# Autodesk Inventor assembly: mini Cryostat FOOT3
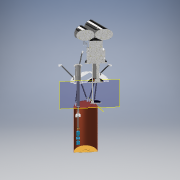
[picture p0: Inventor's stored thumbnail of the model, 180x180]
Saved by Autodesk Inventor 2018 (Build 220112000, 112)
## iProperties
Created: 2018-10-10
Part Number: mini Cryostat FOOT3
Document SubType Name: Assembly
Designer: Admin
Author: Admin
## Documents named in this file (11)
- C:\Users\Admin\Documents\Cryostat\CAD\mini Cryostat FOOT3.iam
- C:\Users\Admin\Documents\Cryostat\CAD\External Models\CH40415 24JUL14 C.ipt
- C:\Users\Admin\Documents\Cryostat\CAD\vacuum jacket long.ipt
- C:\Users\Admin\Documents\Cryostat\CAD\vacuum jacket.ipt
- C:\Users\Admin\Documents\Cryostat\CAD\Top Plate V2.2.ipt
- C:\Users\Admin\Documents\Cryostat\CAD\mini 55K stage.ipt
- C:\Users\Admin\Documents\Cryostat\CAD\foot type 3.iam
- C:\Users\Admin\Documents\Cryostat\CAD\Radiation Sheild 2K.ipt
- C:\Users\Admin\Documents\Cryostat\CAD\still pipe.iam
- C:\Users\Admin\Documents\Cryostat\CAD\4K shield2.iam
- C:\Users\Admin\Documents\Cryostat\CAD\2K8 FEET long.iam
## Components (24 placed, 10 different names)
1. Top Plate V2.2:1 — Mate:16, Mate:18, Mate:19, Mate:20, Mate:21, Mate:26, Mate:135, Mate:136, Mate:137, Mate:138, Mate:139, Mate:140, Mate:141, Mate:142, Mate:143, Mate:144, Mate:145, Mate:146, Mate:149, Mate:150, Mate:153, Mate:154, Mate:155, Mate:156
2. CH40415 24JUL14 C:1 — Mate:16, Mate:18, Mate:26, Mate:161, Mate:195, Mate:197
3. vacuum jacket long:1 — Mate:7, Mate:8, Mate:9
4. vacuum jacket:1 — Mate:7, Mate:8, Mate:9, Mate:19, Mate:20, Mate:21
5. mini 55K stage:1 — Mate:100, Mate:102, Mate:147, Mate:148, Mate:151, Mate:152, Mate:157, Mate:158, Mate:159, Mate:160, Mate:161, Mate:162, Mate:163, Mate:164, Mate:165, Mate:166, Mate:167, Mate:168, Mate:169, Mate:170, Mate:200, Mate:201, Mate:208, Mate:209, Mate:214, Mate:216, Mate:217, Mate:218, Mate:227, Mate:229, Mate:230, Mate:231, Mate:232, Mate:233, Mate:234, Mate:235, Symmetry:1
6. Radiation Sheild 2K:1 — Mate:100, Mate:102
7. still pipe:1 [sub-assembly] — Mate:135, Mate:136, Mate:162, Mate:196
8. foot type 3:1 [sub-assembly] — Mate:143, Mate:155, Mate:158, Mate:164
9. foot type 3:2 [sub-assembly] — Mate:140, Mate:153, Mate:159, Mate:169
10. foot type 3:3 [sub-assembly] — Mate:138, Mate:149, Mate:151, Mate:163
11. foot type 3:4 [sub-assembly] — Mate:144, Mate:154, Mate:160, Mate:168
12. foot type 3:5 [sub-assembly] — Mate:139, Mate:150, Mate:152, Mate:170
13. foot type 3:6 [sub-assembly] — Mate:137, Mate:145, Mate:148, Mate:166
14. foot type 3:7 [sub-assembly] — Mate:141, Mate:156, Mate:157, Mate:165
15. foot type 3:8 [sub-assembly] — Mate:142, Mate:146, Mate:147, Mate:167
16. 4K shield2:1 [sub-assembly] — Mate:195, Mate:196, Mate:197, Mate:198, Mate:202, Mate:203, Mate:204, Mate:210, Mate:211, Mate:212, Mate:213, Mate:219, Mate:220, Mate:221, Mate:222, Mate:223, Mate:224, Mate:225, Mate:226
17. 2K8 FEET long:1 [sub-assembly] — Mate:198, Mate:200, Mate:201, Mate:211
18. 2K8 FEET long:2 [sub-assembly] — Mate:203, Mate:213, Mate:214, Mate:216
19. 2K8 FEET long:3 [sub-assembly] — Mate:204, Mate:212, Mate:217, Mate:218, Symmetry:1
20. 2K8 FEET long:4 [sub-assembly] — Mate:202, Mate:208, Mate:209, Mate:210
21. 2K8 FEET long:5 [sub-assembly] — Mate:222, Mate:226, Mate:227, Mate:230
22. 2K8 FEET long:6 [sub-assembly] — Mate:221, Mate:225, Mate:229, Mate:235
23. 2K8 FEET long:7 [sub-assembly] — Mate:220, Mate:224, Mate:232, Mate:233
24. 2K8 FEET long:8 [sub-assembly] — Mate:219, Mate:223, Mate:231, Mate:234
## Relationships (83: Mate 82, Symmetry 1)
- Mate:7: vacuum jacket long:1 ↔ vacuum jacket:1
- Mate:8: vacuum jacket long:1 ↔ vacuum jacket:1
- Mate:9: vacuum jacket long:1 ↔ vacuum jacket:1
- Mate:16: Top Plate V2.2:1 ↔ CH40415 24JUL14 C:1
- Mate:18: Top Plate V2.2:1 ↔ CH40415 24JUL14 C:1
- Mate:19: Top Plate V2.2:1 ↔ vacuum jacket:1
- Mate:20: Top Plate V2.2:1 ↔ vacuum jacket:1
- Mate:21: Top Plate V2.2:1 ↔ vacuum jacket:1
- Mate:26: Top Plate V2.2:1 ↔ CH40415 24JUL14 C:1
- Mate:100: mini 55K stage:1 ↔ Radiation Sheild 2K:1
- Mate:102: mini 55K stage:1 ↔ Radiation Sheild 2K:1
- Mate:135: Top Plate V2.2:1 ↔ still pipe:1
- Mate:136: Top Plate V2.2:1 ↔ still pipe:1
- Mate:137: Top Plate V2.2:1 ↔ foot type 3:6
- Mate:138: Top Plate V2.2:1 ↔ foot type 3:3
- Mate:139: Top Plate V2.2:1 ↔ foot type 3:5
- Mate:140: Top Plate V2.2:1 ↔ foot type 3:2
- Mate:141: Top Plate V2.2:1 ↔ foot type 3:7
- Mate:142: Top Plate V2.2:1 ↔ foot type 3:8
- Mate:143: Top Plate V2.2:1 ↔ foot type 3:1
- Mate:144: Top Plate V2.2:1 ↔ foot type 3:4
- Mate:145: Top Plate V2.2:1 ↔ foot type 3:6
- Mate:146: Top Plate V2.2:1 ↔ foot type 3:8
- Mate:147: mini 55K stage:1 ↔ foot type 3:8
- Mate:148: mini 55K stage:1 ↔ foot type 3:6
- Mate:149: Top Plate V2.2:1 ↔ foot type 3:3
- Mate:150: Top Plate V2.2:1 ↔ foot type 3:5
- Mate:151: mini 55K stage:1 ↔ foot type 3:3
- Mate:152: mini 55K stage:1 ↔ foot type 3:5
- Mate:153: Top Plate V2.2:1 ↔ foot type 3:2
- Mate:154: Top Plate V2.2:1 ↔ foot type 3:4
- Mate:155: Top Plate V2.2:1 ↔ foot type 3:1
- Mate:156: Top Plate V2.2:1 ↔ foot type 3:7
- Mate:157: mini 55K stage:1 ↔ foot type 3:7
- Mate:158: mini 55K stage:1 ↔ foot type 3:1
- Mate:159: mini 55K stage:1 ↔ foot type 3:2
- Mate:160: mini 55K stage:1 ↔ foot type 3:4
- Mate:161: CH40415 24JUL14 C:1 ↔ mini 55K stage:1
- Mate:162: mini 55K stage:1 ↔ still pipe:1
- Mate:163: mini 55K stage:1 ↔ foot type 3:3
- Mate:164: mini 55K stage:1 ↔ foot type 3:1
- Mate:165: mini 55K stage:1 ↔ foot type 3:7
- Mate:166: mini 55K stage:1 ↔ foot type 3:6
- Mate:167: mini 55K stage:1 ↔ foot type 3:8
- Mate:168: mini 55K stage:1 ↔ foot type 3:4
- Mate:169: mini 55K stage:1 ↔ foot type 3:2
- Mate:170: mini 55K stage:1 ↔ foot type 3:5
- Mate:195: CH40415 24JUL14 C:1 ↔ 4K shield2:1
- Mate:196: still pipe:1 ↔ 4K shield2:1
- Mate:197 (31.75 mm): CH40415 24JUL14 C:1 ↔ 4K shield2:1
- Mate:198: 4K shield2:1 ↔ 2K8 FEET long:1
- Mate:200: mini 55K stage:1 ↔ 2K8 FEET long:1
- Mate:201: mini 55K stage:1 ↔ 2K8 FEET long:1
- Mate:202: 4K shield2:1 ↔ 2K8 FEET long:4
- Mate:203: 4K shield2:1 ↔ 2K8 FEET long:2
- Mate:204: 4K shield2:1 ↔ 2K8 FEET long:3
- Mate:208: mini 55K stage:1 ↔ 2K8 FEET long:4
- Mate:209: mini 55K stage:1 ↔ 2K8 FEET long:4
- Mate:210: 4K shield2:1 ↔ 2K8 FEET long:4
- Mate:211: 4K shield2:1 ↔ 2K8 FEET long:1
- Mate:212: 4K shield2:1 ↔ 2K8 FEET long:3
- Mate:213: 4K shield2:1 ↔ 2K8 FEET long:2
- Mate:214: mini 55K stage:1 ↔ 2K8 FEET long:2
- Mate:216: mini 55K stage:1 ↔ 2K8 FEET long:2
- Mate:217: mini 55K stage:1 ↔ 2K8 FEET long:3
- Mate:218: mini 55K stage:1 ↔ 2K8 FEET long:3
- Mate:219: 4K shield2:1 ↔ 2K8 FEET long:8
- Mate:220: 4K shield2:1 ↔ 2K8 FEET long:7
- Mate:221: 4K shield2:1 ↔ 2K8 FEET long:6
- Mate:222: 4K shield2:1 ↔ 2K8 FEET long:5
- Mate:223: 4K shield2:1 ↔ 2K8 FEET long:8
- Mate:224: 4K shield2:1 ↔ 2K8 FEET long:7
- Mate:225: 4K shield2:1 ↔ 2K8 FEET long:6
- Mate:226: 4K shield2:1 ↔ 2K8 FEET long:5
- Mate:227: mini 55K stage:1 ↔ 2K8 FEET long:5
- Mate:229: mini 55K stage:1 ↔ 2K8 FEET long:6
- Mate:230: mini 55K stage:1 ↔ 2K8 FEET long:5
- Mate:231: mini 55K stage:1 ↔ 2K8 FEET long:8
- Mate:232: mini 55K stage:1 ↔ 2K8 FEET long:7
- Mate:233: mini 55K stage:1 ↔ 2K8 FEET long:7
- Mate:234: mini 55K stage:1 ↔ 2K8 FEET long:8
- Mate:235: mini 55K stage:1 ↔ 2K8 FEET long:6
- Symmetry:1: mini 55K stage:1 ↔ 2K8 FEET long:3
